# Autodesk Inventor assembly: Framing_For_Second_Floor_Window
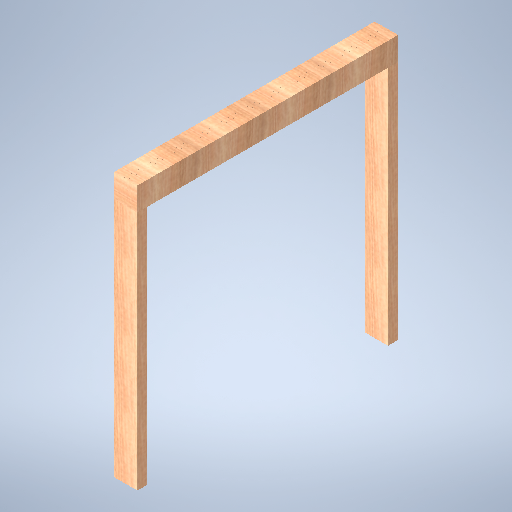
[picture p0: Inventor's stored thumbnail of the model, 512x512]
Saved by Autodesk Inventor 2025.1 (Build 291241020, 241B)
## iProperties
Created: 2024-09-15
Part Number: Framing_For_Second_Floor_Window
Document SubType Name: Assembly
Designer: Tom
Author: Tom
## Documents named in this file (3)
- C:\Users\Tom\Documents\Inventor\Mobility\Additional_Building\Framing_For_Second_Floor_Window.iam
- C:\Users\Tom\Documents\Inventor\Mobility\Additional_Building\Header_With_Dimensions_3.5_x_3.5_x_39_Inches.iam
- C:\Users\Tom\Documents\Inventor\Mobility\Additional_Building\Stud_With_Height_36_Inches.ipt
## Components (3 placed, 2 different names)
1. Header_With_Dimensions_3.5_x_3.5_x_39_Inches:1 [sub-assembly] — Mate:4, Flush:4, Flush:5
2. Stud_With_Height_36_Inches:1 — Mate:1, Mate:2, Mate:3, Flush:1, Flush:2, Flush:3, Mate:4, Flush:4, Flush:5
3. Stud_With_Height_36_Inches:2 — Mate:3, Flush:1, Flush:2, Flush:3
## Relationships (9: Flush 5, Mate 4)
- Mate:1: Stud_With_Height_36_Inches:1
- Mate:2: Stud_With_Height_36_Inches:1
- Mate:3 (914.4 mm): Stud_With_Height_36_Inches:1 ↔ Stud_With_Height_36_Inches:2
- Flush:1: Stud_With_Height_36_Inches:1 ↔ Stud_With_Height_36_Inches:2
- Flush:2: Stud_With_Height_36_Inches:1 ↔ Stud_With_Height_36_Inches:2
- Flush:3: Stud_With_Height_36_Inches:1 ↔ Stud_With_Height_36_Inches:2
- Mate:4: Header_With_Dimensions_3.5_x_3.5_x_39_Inches:1 ↔ Stud_With_Height_36_Inches:1
- Flush:4: Header_With_Dimensions_3.5_x_3.5_x_39_Inches:1 ↔ Stud_With_Height_36_Inches:1
- Flush:5: Header_With_Dimensions_3.5_x_3.5_x_39_Inches:1 ↔ Stud_With_Height_36_Inches:1
